# Autodesk Inventor assembly: ASSEMBLY_Main
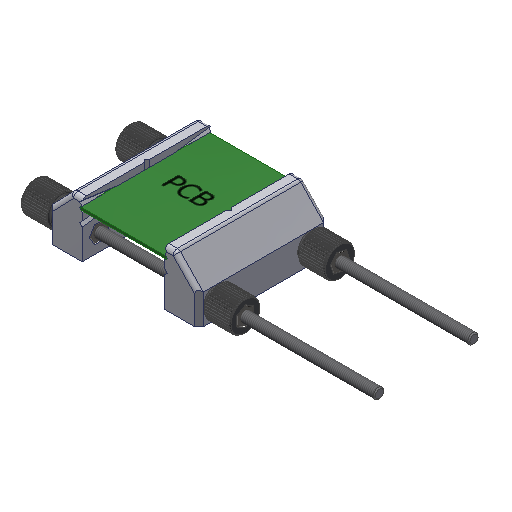
[picture p0: Inventor's stored thumbnail of the model, 512x512]
Saved by Autodesk Inventor 2026.1 (Build 301233000, 233)
## iProperties
Created: 2018-02-17
Part Number: ASSEMBLY_Main
Material: Ogólny
Document SubType Name: Assembly
Designer: Andrzej
Mass: 107.972 g
Surface Area: 445.161 cm^2
Volume: 107.972 cm^3
Density: 1 g/cm^3
Author: Andrzej
## Documents named in this file (8)
- C:\Users\Andrzej\OneDrive\_DRIVE_SYNCH_FILES\__ BYTECHLAB PROJECTS\MECH - 3D Printed PCB Vise\MCAD\1_REV1\ASSEMBLY_MAIN_REVA\ASSEMBLY_Main.iam
- C:\Users\Andrzej\OneDrive\_DRIVE_SYNCH_FILES\__ BYTECHLAB PROJECTS\MECH - 3D Printed PCB Vise\MCAD\1_REV1\ASSEMBLY_MAIN_REVA\3DP_ABS_Jaw_Second_Half.ipt
- C:\Users\Andrzej\OneDrive\_DRIVE_SYNCH_FILES\__ BYTECHLAB PROJECTS\MECH - 3D Printed PCB Vise\MCAD\1_REV1\__COTS_PARTS\COTS_GENERIC_M6_Threaded_Rod_200mm.ipt
- C:\Users\Andrzej\OneDrive\_DRIVE_SYNCH_FILES\__ BYTECHLAB PROJECTS\MECH - 3D Printed PCB Vise\MCAD\1_REV1\ASSEMBLY_MAIN_REVA\3DP_ABS_Jaw_First_Half.ipt
- C:\Users\Andrzej\OneDrive\_DRIVE_SYNCH_FILES\__ BYTECHLAB PROJECTS\MECH - 3D Printed PCB Vise\MCAD\1_REV1\__COTS_PARTS\COTS_GENERIC_M6_Nut.ipt
- C:\Users\Andrzej\OneDrive\_DRIVE_SYNCH_FILES\__ BYTECHLAB PROJECTS\MECH - 3D Printed PCB Vise\MCAD\1_REV1\ASSEMBLY_MAIN_REVA\ASSEMBLY_Nut_Knob.iam
- C:\Users\Andrzej\OneDrive\_DRIVE_SYNCH_FILES\__ BYTECHLAB PROJECTS\MECH - 3D Printed PCB Vise\MCAD\1_REV1\__COTS_PARTS\COTS_GENERIC_PCB.ipt
- C:\Users\Andrzej\OneDrive\_DRIVE_SYNCH_FILES\__ BYTECHLAB PROJECTS\MECH - 3D Printed PCB Vise\MCAD\1_REV1\__COTS_PARTS\COTS_GENERIC_10x4mm_Neodymium_Magnet.ipt
## Components (13 placed, 7 different names)
1. 3DP_ABS_Jaw_Second_Half:1 — Zestawiający:2, Zestawiający:3, Zestawiający:4, Równoległy:1, Równoległy:2, Zestawiający:13, Zestawiający:14, Mate:20, Mate:22
2. 3DP_ABS_Jaw_First_Half:1 — Zestawiający:4, Równoległy:1, Równoległy:2, Zestawiający:5, Zestawiający:7, Zestawiający:8, Zestawiający:9, Zestawiający:11, Zestawiający:12, Równoległy:5, Równoległy:6, Mate:19, Mate:21
3. ASSEMBLY_Nut_Knob:1 [sub-assembly] — Zestawiający:11, Zestawiający:17, Równoległy:4
4. ASSEMBLY_Nut_Knob:2 [sub-assembly] — Zestawiający:14, Zestawiający:16
5. ASSEMBLY_Nut_Knob:3 [sub-assembly] — Zestawiający:13, Zestawiający:15
6. ASSEMBLY_Nut_Knob:4 [sub-assembly] — Zestawiający:12, Zestawiający:18, Równoległy:3
7. COTS_GENERIC_PCB:1 — Równoległy:5, Równoległy:6
8. COTS_GENERIC_10x4mm_Neodymium_Magnet:1 — Mate:19, Mate:21
9. COTS_GENERIC_10x4mm_Neodymium_Magnet:2 — Mate:20, Mate:22
10. COTS_GENERIC_M6_Nut:2 — Zestawiający:8, Zestawiający:9, Zestawiający:10
11. COTS_GENERIC_M6_Nut:1 — Zestawiający:5, Zestawiający:6, Zestawiający:7
12. COTS_GENERIC_M6_Threaded_Rod_200mm:2 — Zestawiający:2, Zestawiający:10, Zestawiający:15, Zestawiający:17, Równoległy:4
13. COTS_GENERIC_M6_Threaded_Rod_200mm:1 — Zestawiający:3, Zestawiający:6, Zestawiający:16, Zestawiający:18, Równoległy:3
## Relationships (27: Mate 21, Flush 6)
- Zestawiający:2 [Mate]: 3DP_ABS_Jaw_Second_Half:1 ↔ COTS_GENERIC_M6_Threaded_Rod_200mm:2
- Zestawiający:3 [Mate]: 3DP_ABS_Jaw_Second_Half:1 ↔ COTS_GENERIC_M6_Threaded_Rod_200mm:1
- Zestawiający:4 [Mate] (48 mm): 3DP_ABS_Jaw_Second_Half:1 ↔ 3DP_ABS_Jaw_First_Half:1
- Równoległy:1 [Flush]: 3DP_ABS_Jaw_Second_Half:1 ↔ 3DP_ABS_Jaw_First_Half:1
- Równoległy:2 [Flush]: 3DP_ABS_Jaw_Second_Half:1 ↔ 3DP_ABS_Jaw_First_Half:1
- Zestawiający:5 [Mate]: 3DP_ABS_Jaw_First_Half:1 ↔ COTS_GENERIC_M6_Nut:1
- Zestawiający:6 [Mate]: COTS_GENERIC_M6_Nut:1 ↔ COTS_GENERIC_M6_Threaded_Rod_200mm:1
- Zestawiający:7 [Mate]: 3DP_ABS_Jaw_First_Half:1 ↔ COTS_GENERIC_M6_Nut:1
- Zestawiający:8 [Mate]: 3DP_ABS_Jaw_First_Half:1 ↔ COTS_GENERIC_M6_Nut:2
- Zestawiający:9 [Mate]: 3DP_ABS_Jaw_First_Half:1 ↔ COTS_GENERIC_M6_Nut:2
- Zestawiający:10 [Mate]: COTS_GENERIC_M6_Nut:2 ↔ COTS_GENERIC_M6_Threaded_Rod_200mm:2
- Zestawiający:11 [Mate]: 3DP_ABS_Jaw_First_Half:1 ↔ ASSEMBLY_Nut_Knob:1
- Zestawiający:12 [Mate]: 3DP_ABS_Jaw_First_Half:1 ↔ ASSEMBLY_Nut_Knob:4
- Zestawiający:13 [Mate]: 3DP_ABS_Jaw_Second_Half:1 ↔ ASSEMBLY_Nut_Knob:3
- Zestawiający:14 [Mate]: 3DP_ABS_Jaw_Second_Half:1 ↔ ASSEMBLY_Nut_Knob:2
- Zestawiający:15 [Mate]: ASSEMBLY_Nut_Knob:3 ↔ COTS_GENERIC_M6_Threaded_Rod_200mm:2
- Zestawiający:16 [Mate]: ASSEMBLY_Nut_Knob:2 ↔ COTS_GENERIC_M6_Threaded_Rod_200mm:1
- Zestawiający:17 [Mate]: ASSEMBLY_Nut_Knob:1 ↔ COTS_GENERIC_M6_Threaded_Rod_200mm:2
- Zestawiający:18 [Mate]: ASSEMBLY_Nut_Knob:4 ↔ COTS_GENERIC_M6_Threaded_Rod_200mm:1
- Równoległy:3 [Flush]: ASSEMBLY_Nut_Knob:4 ↔ COTS_GENERIC_M6_Threaded_Rod_200mm:1
- Równoległy:4 [Flush]: ASSEMBLY_Nut_Knob:1 ↔ COTS_GENERIC_M6_Threaded_Rod_200mm:2
- Równoległy:5 [Flush]: 3DP_ABS_Jaw_First_Half:1 ↔ COTS_GENERIC_PCB:1
- Równoległy:6 [Flush] (4.75 mm): 3DP_ABS_Jaw_First_Half:1 ↔ COTS_GENERIC_PCB:1
- Mate:19: 3DP_ABS_Jaw_First_Half:1 ↔ COTS_GENERIC_10x4mm_Neodymium_Magnet:1
- Mate:20: 3DP_ABS_Jaw_Second_Half:1 ↔ COTS_GENERIC_10x4mm_Neodymium_Magnet:2
- Mate:21: 3DP_ABS_Jaw_First_Half:1 ↔ COTS_GENERIC_10x4mm_Neodymium_Magnet:1
- Mate:22: 3DP_ABS_Jaw_Second_Half:1 ↔ COTS_GENERIC_10x4mm_Neodymium_Magnet:2
